# Autodesk Inventor assembly: Сборка2
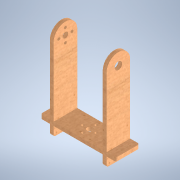
[picture p0: Inventor's stored thumbnail of the model, 180x180]
Saved by Autodesk Inventor 2020.1 (Build 241239000, 239)
## iProperties
Created: 2021-08-12
Part Number: Сборка2
Document SubType Name: Assembly
Designer: Ni3na
Author: Ni3na
## Documents named in this file (4)
- D:\GitHub\avatar-kvantoriada\3D\Сборка2.iam
- D:\GitHub\avatar-kvantoriada\3D\Деталь2.ipt
- D:\GitHub\avatar-kvantoriada\3D\Деталь3.ipt
- D:\GitHub\avatar-kvantoriada\3D\Деталь3_1.ipt
## Components (3 placed, 3 different names)
1. Деталь2:1 — Жесткий:1, Жесткий:2
2. Деталь3:1 — Жесткий:1
3. Деталь3_1:1 — Жесткий:2
## Relationships (2: WeldJoint 2)
- Жесткий:1 [WeldJoint]: Деталь2:1 ↔ Деталь3:1
- Жесткий:2 [WeldJoint]: Деталь2:1 ↔ Деталь3_1:1
